# Autodesk Inventor assembly: Robo_Montado_v3
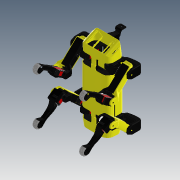
[picture p0: Inventor's stored thumbnail of the model, 180x180]
Saved by Autodesk Inventor 2020 (Build 240168000, 168)
## iProperties
Created: 2022-06-22
Part Number: Robo_Montado_v3
Document SubType Name: Assembly
Designer: JCarlos
Author: JCarlos
## Documents named in this file (8)
- C:\Users\candu\Google Drive\Doutorado_UTFPR\Projeto_1_SpotMicro\Projeto_3D\Robo_Montado_v3\3Dfiles_Q-Robot\Q-Robot.iam
- C:\Users\candu\Google Drive\Doutorado_UTFPR\Projeto_1_SpotMicro\Projeto_3D\Robo_Montado_v3\3Dfiles_Q-Robot\Corpo_Interno_v3.iam
- C:\Users\candu\Google Drive\Doutorado_UTFPR\Projeto_1_SpotMicro\Projeto_3D\Robo_Montado_v3\3Dfiles_Q-Robot\Tronco.iam
- C:\Users\candu\Google Drive\Doutorado_UTFPR\Projeto_1_SpotMicro\Projeto_3D\Robo_Montado_v3\3Dfiles_Q-Robot\Cover_Dianteira.ipt
- C:\Users\candu\Google Drive\Doutorado_UTFPR\Projeto_1_SpotMicro\Projeto_3D\Robo_Montado_v3\3Dfiles_Q-Robot\Cover_Inferior.ipt
- C:\Users\candu\Google Drive\Doutorado_UTFPR\Projeto_1_SpotMicro\Projeto_3D\Robo_Montado_v3\3Dfiles_Q-Robot\Cover_Traseira.ipt
- C:\Users\candu\Google Drive\Doutorado_UTFPR\Projeto_1_SpotMicro\Projeto_3D\Robo_Montado_v3\3Dfiles_Q-Robot\Cover_Superior.ipt
- C:\Users\candu\Google Drive\Doutorado_UTFPR\Projeto_1_SpotMicro\Projeto_3D\Robo_Montado_v3\3Dfiles_Q-Robot\LiDAR.iam
## Components (8 placed, 7 different names)
1. Corpo_Interno_v3:1 [sub-assembly] — Ângulo:1, Ângulo:2, Coincidência:1, Coincidência:2, Coincidência:3, Coincidência:4, Coincidência:5, Coincidência:6
2. Tronco:1 [sub-assembly] — Coincidência:1, Coincidência:2, Coincidência:3, Coincidência:10, Coincidência:11, Coincidência:12
3. Tronco:2 [sub-assembly] — Coincidência:4, Coincidência:5, Coincidência:6, Coincidência:7, Coincidência:8, Coincidência:9, Alinhamento:3
4. Cover_Dianteira:1 — Coincidência:7, Coincidência:8, Coincidência:9, Coincidência:13, Coincidência:16, Coincidência:17, Coincidência:18, Ângulo:3, Alinhamento:1, Ângulo:4, Coincidência:19, Ângulo:5
5. Cover_Inferior:1 — Coincidência:13, Coincidência:14, Coincidência:15
6. Cover_Traseira:1 — Coincidência:10, Coincidência:11, Coincidência:12, Coincidência:14, Coincidência:15
7. Cover_Superior:1 — Coincidência:16, Coincidência:17, Coincidência:18
8. LiDAR:1 [sub-assembly] — Ângulo:3, Alinhamento:1, Ângulo:4, Alinhamento:2
## Relationships (27: Mate 19, Angle 5, Flush 3)
- Ângulo:1 [Angle] (0 deg): Corpo_Interno_v3:1
- Ângulo:2 [Angle] (0 deg): Corpo_Interno_v3:1
- Coincidência:1 [Mate]: Corpo_Interno_v3:1 ↔ Tronco:1
- Coincidência:2 [Mate]: Corpo_Interno_v3:1 ↔ Tronco:1
- Coincidência:3 [Mate]: Corpo_Interno_v3:1 ↔ Tronco:1
- Coincidência:4 [Mate]: Corpo_Interno_v3:1 ↔ Tronco:2
- Coincidência:5 [Mate]: Corpo_Interno_v3:1 ↔ Tronco:2
- Coincidência:6 [Mate]: Corpo_Interno_v3:1 ↔ Tronco:2
- Coincidência:7 [Mate]: Tronco:2 ↔ Cover_Dianteira:1
- Coincidência:8 [Mate]: Tronco:2 ↔ Cover_Dianteira:1
- Coincidência:9 [Mate]: Tronco:2 ↔ Cover_Dianteira:1
- Coincidência:10 [Mate]: Tronco:1 ↔ Cover_Traseira:1
- Coincidência:11 [Mate]: Tronco:1 ↔ Cover_Traseira:1
- Coincidência:12 [Mate]: Tronco:1 ↔ Cover_Traseira:1
- Coincidência:13 [Mate]: Cover_Dianteira:1 ↔ Cover_Inferior:1
- Coincidência:14 [Mate]: Cover_Inferior:1 ↔ Cover_Traseira:1
- Coincidência:15 [Mate]: Cover_Inferior:1 ↔ Cover_Traseira:1
- Coincidência:16 [Mate]: Cover_Dianteira:1 ↔ Cover_Superior:1
- Coincidência:17 [Mate]: Cover_Dianteira:1 ↔ Cover_Superior:1
- Coincidência:18 [Mate]: Cover_Dianteira:1 ↔ Cover_Superior:1
- Ângulo:3 [Angle] (0 deg): Cover_Dianteira:1 ↔ LiDAR:1
- Alinhamento:1 [Flush]: Cover_Dianteira:1 ↔ LiDAR:1
- Ângulo:4 [Angle] (0 deg): Cover_Dianteira:1 ↔ LiDAR:1
- Coincidência:19 [Mate]: Cover_Dianteira:1
- Ângulo:5 [Angle] (-169 deg): Cover_Dianteira:1
- Alinhamento:2 [Flush] (3 mm): LiDAR:1
- Alinhamento:3 [Flush] (-4.5 mm): Tronco:2
